# Autodesk Inventor assembly: 2AM-17-A-1200 - slider
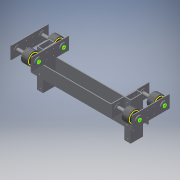
[picture p0: Inventor's stored thumbnail of the model, 180x180]
Saved by Autodesk Inventor 2017 (Build 210142000, 142)
## iProperties
Created: 2017-12-27
Part Number: 2AM-17-A-1200 - slider
Document SubType Name: Assembly
Designer: Micah
Author: Micah
## Documents named in this file (5)
- C:\Users\Micah\Desktop\inventor\CADathon-2017\2AM-17-A-0200 - Smokestack Elevator\2AM-17-A-1200 - moving part.iam
- C:\Users\Micah\Desktop\inventor\CADathon-2017\2AM-17-A-0200 - Smokestack Elevator\2AM-17-P-0203 - moving support.ipt
- C:\Users\Micah\Desktop\inventor\CADathon-2017\2AM-17-A-0200 - Smokestack Elevator\2AM-17-P-0205 - moving structure.ipt
- C:\Users\Micah\Desktop\inventor\CADathon-2017\2AM-17-A-0200 - Smokestack Elevator\2AM-17-A-2200 - slider outside.iam
- C:\Users\Micah\Desktop\inventor\CADathon-2017\2AM-17-A-0200 - Smokestack Elevator\2AM-17-A-4200 - inside slider.iam
## Components (8 placed, 4 different names)
1. 2AM-17-P-0203 - moving support:1 — Mate:2, Mate:3, Insert:1, Insert:2
2. 2AM-17-P-0203 - moving support:2
3. 2AM-17-P-0205 - moving structure:2 — Mate:2, Mate:5
4. 2AM-17-A-2200 - slider outside:1 [sub-assembly] — Mate:4
5. 2AM-17-P-0205 - moving structure:3 — Mate:3, Mate:4
6. 2AM-17-A-2200 - slider outside:2 [sub-assembly] — Mate:5
7. 2AM-17-A-4200 - inside slider:1 [sub-assembly] — Insert:2
8. 2AM-17-A-4200 - inside slider:2 [sub-assembly] — Insert:1
## Relationships (6: Mate 4, Insert 2)
- Mate:2: 2AM-17-P-0203 - moving support:1 ↔ 2AM-17-P-0205 - moving structure:2
- Mate:3: 2AM-17-P-0203 - moving support:1 ↔ 2AM-17-P-0205 - moving structure:3
- Mate:4: 2AM-17-A-2200 - slider outside:1 ↔ 2AM-17-P-0205 - moving structure:3
- Mate:5: 2AM-17-P-0205 - moving structure:2 ↔ 2AM-17-A-2200 - slider outside:2
- Insert:1: 2AM-17-P-0203 - moving support:1 ↔ 2AM-17-A-4200 - inside slider:2
- Insert:2: 2AM-17-P-0203 - moving support:1 ↔ 2AM-17-A-4200 - inside slider:1
